# Autodesk Inventor assembly: 39092
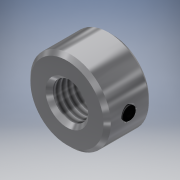
[picture p0: Inventor's stored thumbnail of the model, 180x180]
Saved by Autodesk Inventor 2017.1 (Build 211199000, 199)
## iProperties
Category: Collars
Company: Autodesk Inc.
Created: 2017-01-02
Part Number: 39092
Document SubType Name: Assembly
Designer: Autodesk Inc.
Catalog Web Link: http://www.tetrixrobotics.com/TETRIX_Axle_Set_Collars
Vendor: Tetrix
Author: Autodesk Inc.
## Documents named in this file (3)
- D:\FIRST\FTC KOP 2017\FTC 2017 KOP\Tetrix\Tetrix_39092.iam
- D:\FIRST\FTC KOP 2017\FTC 2017 KOP\Tetrix\Tetrix_739092_Collar.ipt
- D:\FIRST\FTC KOP 2017\FTC 2017 KOP\Tetrix\Tetrix_739092_Screw.ipt
## Components (2 placed, 2 different names)
1. Tetrix_39092_Collar — Mate:1
2. Tetrix_39092_Screw — Mate:1
## Relationships (1: Mate 1)
- Mate:1: Tetrix_39092_Collar ↔ Tetrix_39092_Screw
